# Autodesk Inventor assembly: Gripper_Design_Tendon_v1
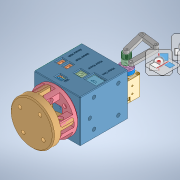
[picture p0: Inventor's stored thumbnail of the model, 180x180]
Saved by Autodesk Inventor 2022 (Build 260153000, 153)
## iProperties
Created: 2021-07-25
Part Number: Gripper_Design_Tendon_v1
Document SubType Name: Assembly
Designer: exllu
Author: exllu
## Documents named in this file (20)
- C:\Users\kylem\OneDrive\Documents\1 - Documents\Gripper Design\Gripper_Design_Tendon_v1.iam
- C:\Users\kylem\OneDrive\Documents\1 - Documents\Gripper Design\Motor_XM,H-430_idler.ipt
- C:\Users\kylem\OneDrive\Documents\1 - Documents\Gripper Design\Pinion_2664N316.ipt
- C:\Users\kylem\OneDrive\Documents\1 - Documents\Gripper Design\Drive_shaft.ipt
- C:\Users\kylem\OneDrive\Documents\1 - Documents\Gripper Design\Motor_horn_mount.ipt
- C:\Users\kylem\OneDrive\Documents\1 - Documents\Gripper Design\Compliant_plate.ipt
- C:\Users\kylem\OneDrive\Documents\1 - Documents\Gripper Design\Finger_mount.ipt
- C:\Users\kylem\OneDrive\Documents\1 - Documents\Gripper Design\UR5_Mounting_Plate.ipt
- C:\Users\kylem\OneDrive\Documents\1 - Documents\Gripper Design\Motor_UR5_mount.ipt
- C:\Users\kylem\OneDrive\Documents\1 - Documents\Gripper Design\U2D2 and Power Board Assembly.iam
- C:\Users\kylem\OneDrive\Documents\1 - Documents\Gripper Design\Contactile Communication Hub.ipt
- C:\Users\kylem\OneDrive\Documents\1 - Documents\Gripper Design\Electronics Box.ipt
- C:\Users\kylem\OneDrive\Documents\1 - Documents\Gripper Design\Electronics Box Lid.ipt
- C:\Users\kylem\OneDrive\Documents\1 - Documents\Gripper Design\Finger Assembly Left.iam
- C:\Users\kylem\OneDrive\Documents\1 - Documents\Gripper Design\Finger Assembly Right.iam
- C:\Users\kylem\OneDrive\Documents\1 - Documents\Gripper Design\IMU_assembly.iam
- C:\Users\kylem\OneDrive\Documents\1 - Documents\Gripper Design\Non_compliant_plate3.ipt
- C:\Users\kylem\OneDrive\Documents\1 - Documents\Gripper Design\Bar.ipt
- C:\Users\kylem\OneDrive\Documents\1 - Documents\Gripper Design\Bar2.ipt
- C:\Users\kylem\OneDrive\Documents\1 - Documents\Gripper Design\Bar3.ipt
## Components (19 placed, 19 different names)
1. Motor_XM,H-430_idler:1 — Flush:1, Flush:2, Flush:3, Mate:15, Mate:16, Mate:264, Flush:54, Mate:270
2. Pinion_2664N316:1 — Mate:20, Mate:21, Mate:265, Mate:266
3. Drive_shaft:1 — Mate:17, Mate:20, Mate:21, Mate:66, Mate:228
4. Motor_horn_mount:1 — Mate:15, Mate:16, Mate:17, Mate:66, Mate:228
5. Compliant_plate:1
6. Finger_mount:2 — Mate:231, Flush:53, Mate:259
7. UR5_Mounting_Plate:1 — Mate:129, Mate:263
8. Motor_UR5_mount:1 — Mate:129, Mate:254, Mate:256, Mate:258, Mate:263
9. U2D2 and Power Board Assembly:1 [sub-assembly] — Flush:49, Mate:216, Mate:218, Flush:51
10. Contactile Communication Hub:1 — Flush:49, Mate:220, Mate:260
11. Electronics Box:1 — Mate:216, Mate:218, Mate:219, Mate:220, Flush:51, Mate:251, Mate:253, Mate:254, Mate:255, Mate:256, Mate:258, Mate:261, Mate:262, Mate:264, Flush:54
12. Electronics Box Lid:1 — Mate:219, Mate:260, Mate:261, Mate:262
13. Finger Assembly Right:1 [sub-assembly] — Mate:231, Flush:53, Mate:259
14. Finger Assembly Left:1 [sub-assembly]
15. IMU_assembly:1 [sub-assembly] — Mate:251, Mate:253, Mate:255
16. Non_compliant_plate3:1
17. Bar:2 — Mate:265, Mate:266, Mate:268, Mate:269, Mate:271, Flush:55
18. Bar2:2 — Mate:268, Mate:269, Mate:270, Mate:272
19. Bar3:1 — Mate:271, Flush:55, Mate:272
## Relationships (40: Mate 32, Flush 8)
- Flush:1: Motor_XM,H-430_idler:1
- Flush:2: Motor_XM,H-430_idler:1
- Flush:3: Motor_XM,H-430_idler:1
- Mate:15: Motor_XM,H-430_idler:1 ↔ Motor_horn_mount:1
- Mate:16: Motor_XM,H-430_idler:1 ↔ Motor_horn_mount:1
- Mate:17: Drive_shaft:1 ↔ Motor_horn_mount:1
- Mate:20: Pinion_2664N316:1 ↔ Drive_shaft:1
- Mate:21: Pinion_2664N316:1 ↔ Drive_shaft:1
- Mate:66: Drive_shaft:1 ↔ Motor_horn_mount:1
- Mate:129: UR5_Mounting_Plate:1 ↔ Motor_UR5_mount:1
- Flush:49 (-1 mm): U2D2 and Power Board Assembly:1 ↔ Contactile Communication Hub:1
- Mate:216 (9 mm): U2D2 and Power Board Assembly:1 ↔ Electronics Box:1
- Mate:218 (1 mm): U2D2 and Power Board Assembly:1 ↔ Electronics Box:1
- Mate:219: Electronics Box:1 ↔ Electronics Box Lid:1
- Mate:220 (1 mm): Contactile Communication Hub:1 ↔ Electronics Box:1
- Flush:51 (2 mm): U2D2 and Power Board Assembly:1 ↔ Electronics Box:1
- Mate:228: Drive_shaft:1 ↔ Motor_horn_mount:1
- Mate:231: Finger_mount:2 ↔ Finger Assembly Right:1
- Flush:53: Finger_mount:2 ↔ Finger Assembly Right:1
- Mate:251: Electronics Box:1 ↔ IMU_assembly:1
- Mate:253: Electronics Box:1 ↔ IMU_assembly:1
- Mate:254: Motor_UR5_mount:1 ↔ Electronics Box:1
- Mate:255: Electronics Box:1 ↔ IMU_assembly:1
- Mate:256: Motor_UR5_mount:1 ↔ Electronics Box:1
- Mate:258: Motor_UR5_mount:1 ↔ Electronics Box:1
- Mate:259: Finger_mount:2 ↔ Finger Assembly Right:1
- Mate:260: Contactile Communication Hub:1 ↔ Electronics Box Lid:1
- Mate:261: Electronics Box:1 ↔ Electronics Box Lid:1
- Mate:262: Electronics Box:1 ↔ Electronics Box Lid:1
- Mate:263: UR5_Mounting_Plate:1 ↔ Motor_UR5_mount:1
- Mate:264: Motor_XM,H-430_idler:1 ↔ Electronics Box:1
- Flush:54: Motor_XM,H-430_idler:1 ↔ Electronics Box:1
- Mate:265: Pinion_2664N316:1 ↔ Bar:2
- Mate:266: Pinion_2664N316:1 ↔ Bar:2
- Mate:268 (20 mm): Bar:2 ↔ Bar2:2
- Mate:269: Bar:2 ↔ Bar2:2
- Mate:270 (-32 mm): Motor_XM,H-430_idler:1 ↔ Bar2:2
- Mate:271: Bar:2 ↔ Bar3:1
- Flush:55: Bar:2 ↔ Bar3:1
- Mate:272: Bar2:2 ↔ Bar3:1
